# Autodesk Inventor assembly: R-H v20
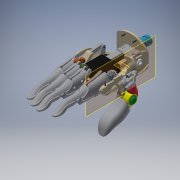
[picture p0: Inventor's stored thumbnail of the model, 180x180]
Saved by Autodesk Inventor 2018 (Build 220112000, 112)
## iProperties
Created: 2017-09-22
Part Number: R-H v20
Material: 一般
Document SubType Name: Assembly
Designer: sktom
Author: sktom
## Documents named in this file (39)
- D:\cloudstrage\NextCloud\Cad_mechanical\HACKberry_SizeM\3Dmodel\R\M-R-H\M-R-H.iam
- D:\cloudstrage\NextCloud\Cad_mechanical\HACKberry_SizeM\3Dmodel\R\M-R-H\M-R-H-01.ipt
- D:\cloudstrage\NextCloud\Cad_mechanical\HACKberry_SizeM\3Dmodel\R\M-R-H\M-R-H-02.ipt
- D:\cloudstrage\NextCloud\Cad_mechanical\HACKberry_SizeM\3Dmodel\R\M-R-H\M-R-H-03.ipt
- D:\cloudstrage\NextCloud\Cad_mechanical\HACKberry_SizeM\3Dmodel\R\M-R-H\M-R-H-04.ipt
- D:\cloudstrage\NextCloud\Cad_mechanical\HACKberry_SizeM\3Dmodel\R\M-R-H\M-R-I\M-R-I .iam
- D:\cloudstrage\NextCloud\Cad_mechanical\HACKberry_SizeM\3Dmodel\R\M-R-H\M-R-O\M-R-O.iam
- D:\cloudstrage\NextCloud\Cad_mechanical\HACKberry_SizeM\3Dmodel\R\M-R-H\M-R-H-05.ipt
- D:\cloudstrage\NextCloud\Cad_mechanical\HACKberry_SizeM\3Dmodel\R\M-R-H\M-R-H-06.ipt
- D:\cloudstrage\NextCloud\Cad_mechanical\HACKberry_SizeM\3Dmodel\R\M-R-H\M-R-H-07.ipt
- D:\cloudstrage\NextCloud\Cad_mechanical\HACKberry_SizeM\3Dmodel\R\M-R-H\M-R-H-08.ipt
- D:\cloudstrage\NextCloud\Cad_mechanical\HACKberry_SizeM\3Dmodel\R\M-R-H\M-R-H-15.ipt
- D:\cloudstrage\NextCloud\Cad_mechanical\HACKberry_SizeM\3Dmodel\R\M-R-H\M-R-H-10.ipt
- D:\cloudstrage\NextCloud\Cad_mechanical\HACKberry_SizeM\3Dmodel\R\M-R-H\M-R-H-11.ipt
- D:\cloudstrage\NextCloud\Cad_mechanical\HACKberry_SizeM\3Dmodel\R\M-R-H\M-R-H-12.ipt
- D:\cloudstrage\NextCloud\Cad_mechanical\HACKberry_SizeM\3Dmodel\R\M-R-H\M-R-H-13.ipt
- D:\cloudstrage\NextCloud\Cad_mechanical\HACKberry_SizeM\3Dmodel\R\M-R-H\M-R-H-14.ipt
- D:\cloudstrage\NextCloud\Cad_mechanical\HACKberry_SizeM\3Dmodel\R\M-R-H\M-R-T\M-R-T.iam
- D:\cloudstrage\NextCloud\Cad_mechanical\HACKberry_SizeM\3Dmodel\R\M-R-H\FL674ZZ.ipt
- D:\cloudstrage\NextCloud\Cad_mechanical\HACKberry_SizeM\3Dmodel\R\M-R-H\GWS_Micro2BBMG.ipt
- D:\cloudstrage\NextCloud\Cad_mechanical\HACKberry_SizeM\3Dmodel\R\M-R-H\Servo_HK282A_Hone.ipt
- D:\cloudstrage\NextCloud\Cad_mechanical\HACKberry_SizeM\3Dmodel\R\M-R-H\MetalCollarPh3L4.5.ipt
- D:\cloudstrage\NextCloud\Cad_mechanical\HACKberry_SizeM\3Dmodel\R\M-R-H\WasherM2Ph4.3T0 v1.ipt
- D:\cloudstrage\NextCloud\Cad_mechanical\HACKberry_SizeM\3Dmodel\R\M-R-H\ASV-15MG.ipt
- D:\cloudstrage\NextCloud\Cad_mechanical\HACKberry_SizeM\3Dmodel\R\M-R-H\ASV-15MGSingleHorn01.ipt
- D:\cloudstrage\NextCloud\Cad_mechanical\HACKberry_SizeM\3Dmodel\R\M-R-H\MotorHolder_forM.ipt
- D:\cloudstrage\NextCloud\Cad_mechanical\HACKberry_SizeM\3Dmodel\R\M-R-H\Dummy_PCB.ipt
- D:\cloudstrage\NextCloud\Cad_mechanical\HACKberry_SizeM\3Dmodel\R\M-R-H\MJ074N.ipt
- D:\cloudstrage\NextCloud\Cad_mechanical\HACKberry_SizeM\3Dmodel\R\M-R-H\MJ179PH.ipt
- D:\cloudstrage\NextCloud\Cad_mechanical\HACKberry_SizeM\3Dmodel\R\M-R-H\H3-2.ipt
- D:\cloudstrage\NextCloud\Cad_mechanical\HACKberry_SizeM\3Dmodel\R\M-R-H\530470310.ipt
- D:\cloudstrage\NextCloud\Cad_mechanical\HACKberry_SizeM\3Dmodel\R\M-R-H\SKRPACE010.ipt
- D:\cloudstrage\NextCloud\Cad_mechanical\HACKberry_SizeM\3Dmodel\R\M-R-H\SS-12D00-G5.ipt
- D:\cloudstrage\NextCloud\Cad_mechanical\HACKberry_SizeM\3Dmodel\R\M-R-H\M1.7_L8.ipt
- D:\cloudstrage\NextCloud\Cad_mechanical\HACKberry_SizeM\3Dmodel\R\M-R-H\M2_L8.ipt
- D:\cloudstrage\NextCloud\Cad_mechanical\HACKberry_SizeM\3Dmodel\R\M-R-H\M2_L6.ipt
- D:\cloudstrage\NextCloud\Cad_mechanical\HACKberry_SizeM\3Dmodel\R\M-R-H\M3_L6.ipt
- D:\cloudstrage\NextCloud\Cad_mechanical\HACKberry_SizeM\3Dmodel\R\M-R-H\Pololu_A_Star_32U4_Micro.ipt
- D:\cloudstrage\NextCloud\Cad_mechanical\HACKberry_SizeM\3Dmodel\R\M-R-H\GWS_Micro2BBMG_hone.ipt
## Components (74 placed, 38 different names)
1. R-H-01 v1:1 — 挿入:61, 挿入:62
2. R-H-02 v1:1 — 挿入:3, 回転:1, 回転:2, 角度:1, 挿入:5, 挿入:7, 挿入:9, 挿入:11, 円柱状:1, メイト:3, メイト:4, フラッシュ:2, 挿入:26, 挿入:27, 挿入:28, 挿入:29, メイト:6, メイト:7, フラッシュ:3, 円柱状:8, 挿入:36, 挿入:37, 挿入:61, 挿入:62
3. R-H-03 v1:1 — 挿入:11, 挿入:30
4. R-H-04 v1:1 — 回転:2, 角度:1, 挿入:31
5. R-I v7:1 [sub-assembly] — 回転:1
6. R-O v4:1 [sub-assembly] — 挿入:5, 挿入:41
7. R-O v4:2 [sub-assembly] — 挿入:9, 回転:3
8. R-O v4:3 [sub-assembly] — 挿入:7, 挿入:42
9. R-H-05 v1:1 — 挿入:21
10. R-H-06 v1:1 — 挿入:22
11. R-H-07 v1:1 — 回転:3, 挿入:24
12. R-H-15 v2:1 — 挿入:27, 挿入:28, メイト:29, メイト:30, メイト:31, 挿入:34, 挿入:35
13. R-H-10 v1:1 — フラッシュ:11, フラッシュ:12, メイト:27
14. R-H-11 v1:1 — フラッシュ:10, フラッシュ:11, フラッシュ:12, フラッシュ:13, メイト:27, メイト:28, メイト:31
15. R-H-12 v1:1 — フラッシュ:10, フラッシュ:13, メイト:28
16. R-H-13 v1:1 — メイト:29
17. R-H-14 v1:1 — メイト:30
18. FL674ZZ:1 — 挿入:3, 挿入:38
19. GWS_Micro2BBMG:1 — 円柱状:1, 挿入:58, 挿入:59, 挿入:63
20. Servo_HK282A_Hone:1 — 円柱状:8, 挿入:32, 挿入:33
21. MetalCollarPh3L4.5:1 — 挿入:17
22. MetalCollarPh3L4.5:2 — 挿入:18
23. MetalCollarPh3L4.5:3 — 挿入:20
24. MetalCollarPh3L4.5:4 — 挿入:19
25. WasherM2Ph4.3T0 v1:1 — 挿入:19, 挿入:48
26. WasherM2Ph4.3T0 v1:2 — 挿入:17, 挿入:22, 挿入:51
27. WasherM2Ph4.3T0 v1:3 — 挿入:20, 挿入:21, 挿入:49
28. WasherM2Ph4.3T0 v1:4 — 挿入:18, 挿入:50
29. ASV-15MG:1 — 挿入:23, メイト:3, メイト:4
30. ASV-15MGSingleHorn01:1 — 挿入:23, 挿入:25
31. MetalCollarPh3L4.5:5 — 挿入:24, 挿入:25, 挿入:46
32. MotorHolder_forM:1 — フラッシュ:2, 挿入:52, 挿入:53, 挿入:54, 挿入:55, 挿入:56, 挿入:57
33. Dummy_PCB:1 — 挿入:26, メイト:5, メイト:8, フラッシュ:4, フラッシュ:5, メイト:9, メイト:10, メイト:12, メイト:13, メイト:14, メイト:15, メイト:16, メイト:17, メイト:18, メイト:19, メイト:20, メイト:21, メイト:22, メイト:23, メイト:24, メイト:25, メイト:26, フラッシュ:14, メイト:32, フラッシュ:15
34. MJ074N:1 — 挿入:29
35. MJ179PH:1 — メイト:5, メイト:6, メイト:7, フラッシュ:3
36. H3-2:1 — メイト:8, フラッシュ:4, フラッシュ:5, フラッシュ:6, フラッシュ:7
37. H3-2:2 — メイト:9, フラッシュ:6, フラッシュ:7, フラッシュ:8, フラッシュ:9
38. 530470310:1 — メイト:10, フラッシュ:8, フラッシュ:9
39. SKRPACE010:1 — メイト:12, メイト:14, メイト:15
40. SS-12D00-G5:1 — メイト:13, メイト:22, メイト:23
41. SKRPACE010:2 — メイト:16, メイト:17, メイト:18
42. SKRPACE010:3 — メイト:19, メイト:20, メイト:21
43. SKRPACE010:4 — メイト:24, メイト:25, メイト:26
44. M1.7_L8:1 — 挿入:31
45. M1.7_L8:2 — 挿入:30
46. M1.7_L8:3 — 挿入:33
47. M1.7_L8:4 — 挿入:32
48. M1.7_L8:5 — 挿入:34
49. M1.7_L8:6 — 挿入:35
50. M1.7_L8:7 — 挿入:36
51. M1.7_L8:8 — 挿入:37
52. M-R-T:1 [sub-assembly] — 挿入:38
53. MetalCollarPh3L4.5:6 — 挿入:41
54. MetalCollarPh3L4.5:7 — 挿入:42
55. M2_L8:3
56. M2_L8:4
57. M2_L8:5
58. WasherM2Ph4.3T0 v1:5 — 挿入:46, 挿入:47
59. M2_L8:6 — 挿入:47
60. M2_L8:7 — 挿入:48
61. M2_L8:8 — 挿入:49
62. M2_L8:9 — 挿入:50
63. M2_L8:10 — 挿入:51
64. M2_L8:11 — 挿入:53
65. M2_L8:12 — 挿入:52
66. M2_L6:1 — 挿入:54
67. M2_L6:2 — 挿入:55
68. M2_L6:3 — 挿入:56
69. M2_L6:4 — 挿入:57
70. M3_L6:1 — 挿入:58
71. M3_L6:2 — 挿入:59
72. Pololu_A_Star_32U4_Micro:1 — フラッシュ:14, メイト:32, フラッシュ:15
73. GWS_Micro2BBMG_hone:1 — 挿入:63, 挿入:64, 挿入:65
74. 平歯車1:1 — 挿入:64, 挿入:65
## Relationships (97: Insert 48, Mate 29, Flush 14, RevoluteJoint 3, CylindricalJoint 2, Angle 1)
- 挿入:3 [Insert]: R-H-02 v1:1 ↔ FL674ZZ:1
- 回転:1 [RevoluteJoint] (0.1 mm): R-H-02 v1:1 ↔ R-I v7:1
- 回転:2 [RevoluteJoint]: R-H-02 v1:1 ↔ R-H-04 v1:1
- 角度:1 [Angle] (179.9087 deg): R-H-02 v1:1 ↔ R-H-04 v1:1
- 挿入:5 [Insert] (0.1 mm): R-H-02 v1:1 ↔ R-O v4:1
- 挿入:7 [Insert] (0.1 mm): R-H-02 v1:1 ↔ R-O v4:3
- 挿入:9 [Insert] (0.1 mm): R-H-02 v1:1 ↔ R-O v4:2
- 挿入:11 [Insert]: R-H-02 v1:1 ↔ R-H-03 v1:1
- 円柱状:1 [CylindricalJoint]: R-H-02 v1:1 ↔ GWS_Micro2BBMG:1
- 回転:3 [RevoluteJoint] (-0.5 mm): R-O v4:2 ↔ R-H-07 v1:1
- 挿入:17 [Insert]: MetalCollarPh3L4.5:1 ↔ WasherM2Ph4.3T0 v1:2
- 挿入:18 [Insert]: MetalCollarPh3L4.5:2 ↔ WasherM2Ph4.3T0 v1:4
- 挿入:19 [Insert]: MetalCollarPh3L4.5:4 ↔ WasherM2Ph4.3T0 v1:1
- 挿入:20 [Insert]: MetalCollarPh3L4.5:3 ↔ WasherM2Ph4.3T0 v1:3
- 挿入:21 [Insert]: R-H-05 v1:1 ↔ WasherM2Ph4.3T0 v1:3
- 挿入:22 [Insert]: R-H-06 v1:1 ↔ WasherM2Ph4.3T0 v1:2
- 挿入:23 [Insert]: ASV-15MG:1 ↔ ASV-15MGSingleHorn01:1
- 挿入:24 [Insert]: R-H-07 v1:1 ↔ MetalCollarPh3L4.5:5
- 挿入:25 [Insert]: ASV-15MGSingleHorn01:1 ↔ MetalCollarPh3L4.5:5
- メイト:3 [Mate]: R-H-02 v1:1 ↔ ASV-15MG:1
- メイト:4 [Mate] (3 mm): R-H-02 v1:1 ↔ ASV-15MG:1
- フラッシュ:2 [Flush]: R-H-02 v1:1 ↔ MotorHolder_forM:1
- 挿入:26 [Insert]: R-H-02 v1:1 ↔ Dummy_PCB:1
- 挿入:27 [Insert]: R-H-02 v1:1 ↔ R-H-15 v2:1
- 挿入:28 [Insert]: R-H-02 v1:1 ↔ R-H-15 v2:1
- 挿入:29 [Insert]: R-H-02 v1:1 ↔ MJ074N:1
- メイト:5 [Mate]: Dummy_PCB:1 ↔ MJ179PH:1
- メイト:6 [Mate]: R-H-02 v1:1 ↔ MJ179PH:1
- メイト:7 [Mate] (0.2 mm): R-H-02 v1:1 ↔ MJ179PH:1
- フラッシュ:3 [Flush]: R-H-02 v1:1 ↔ MJ179PH:1
- メイト:8 [Mate]: Dummy_PCB:1 ↔ H3-2:1
- フラッシュ:4 [Flush] (2 mm): Dummy_PCB:1 ↔ H3-2:1
- フラッシュ:5 [Flush] (5.5 mm): Dummy_PCB:1 ↔ H3-2:1
- メイト:9 [Mate]: Dummy_PCB:1 ↔ H3-2:2
- フラッシュ:6 [Flush]: H3-2:1 ↔ H3-2:2
- フラッシュ:7 [Flush] (3.1 mm): H3-2:1 ↔ H3-2:2
- メイト:10 [Mate]: Dummy_PCB:1 ↔ 530470310:1
- フラッシュ:8 [Flush] (3.1 mm): H3-2:2 ↔ 530470310:1
- フラッシュ:9 [Flush]: H3-2:2 ↔ 530470310:1
- メイト:12 [Mate]: Dummy_PCB:1 ↔ SKRPACE010:1
- メイト:13 [Mate]: Dummy_PCB:1 ↔ SS-12D00-G5:1
- メイト:14 [Mate]: Dummy_PCB:1 ↔ SKRPACE010:1
- メイト:15 [Mate]: Dummy_PCB:1 ↔ SKRPACE010:1
- メイト:16 [Mate]: Dummy_PCB:1 ↔ SKRPACE010:2
- メイト:17 [Mate]: Dummy_PCB:1 ↔ SKRPACE010:2
- メイト:18 [Mate]: Dummy_PCB:1 ↔ SKRPACE010:2
- メイト:19 [Mate]: Dummy_PCB:1 ↔ SKRPACE010:3
- メイト:20 [Mate]: Dummy_PCB:1 ↔ SKRPACE010:3
- メイト:21 [Mate]: Dummy_PCB:1 ↔ SKRPACE010:3
- メイト:22 [Mate]: Dummy_PCB:1 ↔ SS-12D00-G5:1
- メイト:23 [Mate]: Dummy_PCB:1 ↔ SS-12D00-G5:1
- メイト:24 [Mate]: Dummy_PCB:1 ↔ SKRPACE010:4
- メイト:25 [Mate]: Dummy_PCB:1 ↔ SKRPACE010:4
- メイト:26 [Mate]: Dummy_PCB:1 ↔ SKRPACE010:4
- フラッシュ:10 [Flush]: R-H-11 v1:1 ↔ R-H-12 v1:1
- フラッシュ:11 [Flush]: R-H-10 v1:1 ↔ R-H-11 v1:1
- フラッシュ:12 [Flush]: R-H-10 v1:1 ↔ R-H-11 v1:1
- フラッシュ:13 [Flush]: R-H-11 v1:1 ↔ R-H-12 v1:1
- メイト:27 [Mate] (0.2 mm): R-H-10 v1:1 ↔ R-H-11 v1:1
- メイト:28 [Mate] (0.2 mm): R-H-11 v1:1 ↔ R-H-12 v1:1
- メイト:29 [Mate] (0.35 mm): R-H-15 v2:1 ↔ R-H-13 v1:1
- メイト:30 [Mate] (0.35 mm): R-H-15 v2:1 ↔ R-H-14 v1:1
- メイト:31 [Mate] (0.35 mm): R-H-15 v2:1 ↔ R-H-11 v1:1
- 挿入:30 [Insert]: R-H-03 v1:1 ↔ M1.7_L8:2
- 挿入:31 [Insert]: R-H-04 v1:1 ↔ M1.7_L8:1
- 円柱状:8 [CylindricalJoint]: R-H-02 v1:1 ↔ Servo_HK282A_Hone:1
- 挿入:32 [Insert]: Servo_HK282A_Hone:1 ↔ M1.7_L8:4
- 挿入:33 [Insert]: Servo_HK282A_Hone:1 ↔ M1.7_L8:3
- 挿入:34 [Insert]: R-H-15 v2:1 ↔ M1.7_L8:5
- 挿入:35 [Insert]: R-H-15 v2:1 ↔ M1.7_L8:6
- 挿入:36 [Insert]: R-H-02 v1:1 ↔ M1.7_L8:7
- 挿入:37 [Insert]: R-H-02 v1:1 ↔ M1.7_L8:8
- 挿入:38 [Insert]: FL674ZZ:1 ↔ M-R-T:1
- 挿入:41 [Insert]: R-O v4:1 ↔ MetalCollarPh3L4.5:6
- 挿入:42 [Insert]: R-O v4:3 ↔ MetalCollarPh3L4.5:7
- 挿入:46 [Insert]: MetalCollarPh3L4.5:5 ↔ WasherM2Ph4.3T0 v1:5
- 挿入:47 [Insert]: WasherM2Ph4.3T0 v1:5 ↔ M2_L8:6
- 挿入:48 [Insert]: WasherM2Ph4.3T0 v1:1 ↔ M2_L8:7
- 挿入:49 [Insert]: WasherM2Ph4.3T0 v1:3 ↔ M2_L8:8
- 挿入:50 [Insert]: WasherM2Ph4.3T0 v1:4 ↔ M2_L8:9
- 挿入:51 [Insert]: WasherM2Ph4.3T0 v1:2 ↔ M2_L8:10
- 挿入:52 [Insert]: MotorHolder_forM:1 ↔ M2_L8:12
- 挿入:53 [Insert]: MotorHolder_forM:1 ↔ M2_L8:11
- 挿入:54 [Insert]: MotorHolder_forM:1 ↔ M2_L6:1
- 挿入:55 [Insert]: MotorHolder_forM:1 ↔ M2_L6:2
- 挿入:56 [Insert]: MotorHolder_forM:1 ↔ M2_L6:3
- 挿入:57 [Insert]: MotorHolder_forM:1 ↔ M2_L6:4
- 挿入:58 [Insert]: GWS_Micro2BBMG:1 ↔ M3_L6:1
- 挿入:59 [Insert]: GWS_Micro2BBMG:1 ↔ M3_L6:2
- フラッシュ:14 [Flush]: Dummy_PCB:1 ↔ Pololu_A_Star_32U4_Micro:1
- メイト:32 [Mate] (2 mm): Dummy_PCB:1 ↔ Pololu_A_Star_32U4_Micro:1
- フラッシュ:15 [Flush] (3 mm): Dummy_PCB:1 ↔ Pololu_A_Star_32U4_Micro:1
- 挿入:61 [Insert]: R-H-01 v1:1 ↔ R-H-02 v1:1
- 挿入:62 [Insert]: R-H-01 v1:1 ↔ R-H-02 v1:1
- 挿入:63 [Insert]: GWS_Micro2BBMG:1 ↔ GWS_Micro2BBMG_hone:1
- 挿入:64 [Insert]: GWS_Micro2BBMG_hone:1 ↔ 平歯車1:1
- 挿入:65 [Insert]: GWS_Micro2BBMG_hone:1 ↔ 平歯車1:1
